# Autodesk Inventor assembly: MonsterHolderAssembly
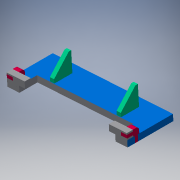
[picture p0: Inventor's stored thumbnail of the model, 180x180]
Saved by Autodesk Inventor 2019 (Build 230136000, 136)
## iProperties
Created: 2018-12-04
Part Number: MonsterHolderAssembly
Document SubType Name: Assembly
Designer: Administrator
Author: Administrator
## Documents named in this file (5)
- H:\Space\Monster Holder\MonsterHolderAssembly.iam
- H:\Space\Monster Holder\MonsterHolderBase.ipt
- H:\Space\Monster Holder\MonsterHolderSupport1.ipt
- H:\Space\Monster Holder\MonsterHolderSupport3.ipt
- H:\Space\Monster Holder\MonsterSupportHolder4.ipt
## Components (7 placed, 4 different names)
1. MonsterHolderBase:1 — Mate:1, Mate:2, Mate:3, Mate:4, Mate:10, Mate:11, Mate:12, Mate:13, Mate:14, Flush:1, Mate:15, Mate:19, Mate:20, Mate:21, Mate:22, Mate:23, Mate:24
2. MonsterHolderSupport1:1 — Mate:1, Mate:2
3. MonsterHolderSupport1:2 — Mate:3, Mate:4
4. MonsterHolderSupport3:1 — Mate:13, Mate:14, Flush:1
5. MonsterHolderSupport3:2 — Mate:10, Mate:11, Mate:12
6. MonsterSupportHolder4:1 — Mate:15, Mate:20, Mate:21, Mate:22
7. MonsterSupportHolder4:2 — Mate:19, Mate:23, Mate:24
## Relationships (17: Mate 16, Flush 1)
- Mate:1: MonsterHolderBase:1 ↔ MonsterHolderSupport1:1
- Mate:2: MonsterHolderBase:1 ↔ MonsterHolderSupport1:1
- Mate:3: MonsterHolderBase:1 ↔ MonsterHolderSupport1:2
- Mate:4: MonsterHolderBase:1 ↔ MonsterHolderSupport1:2
- Mate:10: MonsterHolderBase:1 ↔ MonsterHolderSupport3:2
- Mate:11: MonsterHolderBase:1 ↔ MonsterHolderSupport3:2
- Mate:12: MonsterHolderBase:1 ↔ MonsterHolderSupport3:2
- Mate:13: MonsterHolderBase:1 ↔ MonsterHolderSupport3:1
- Mate:14: MonsterHolderBase:1 ↔ MonsterHolderSupport3:1
- Flush:1: MonsterHolderBase:1 ↔ MonsterHolderSupport3:1
- Mate:15: MonsterHolderBase:1 ↔ MonsterSupportHolder4:1
- Mate:19: MonsterHolderBase:1 ↔ MonsterSupportHolder4:2
- Mate:20: MonsterHolderBase:1 ↔ MonsterSupportHolder4:1
- Mate:21: MonsterHolderBase:1 ↔ MonsterSupportHolder4:1
- Mate:22: MonsterHolderBase:1 ↔ MonsterSupportHolder4:1
- Mate:23: MonsterHolderBase:1 ↔ MonsterSupportHolder4:2
- Mate:24: MonsterHolderBase:1 ↔ MonsterSupportHolder4:2
